# Autodesk Inventor assembly: Sestava
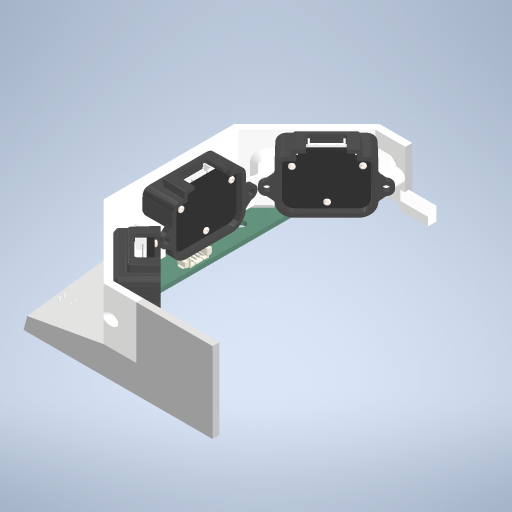
[picture p0: Inventor's stored thumbnail of the model, 512x512]
Saved by Autodesk Inventor 2024 (Build 280153000, 153)
## iProperties
Created: 2024-01-31
Part Number: Sestava
Document SubType Name: Assembly
Designer: Simak
Author: Simak
## Documents named in this file (5)
- C:\Users\Simak\OneDrive\Dokumenty\GitHub\RoboCop\- 3D -\_wip\Sestava.iam
- C:\Users\Simak\OneDrive\Dokumenty\GitHub\RoboCop\- 3D -\_wip\new_plech.ipt
- C:\Users\Simak\OneDrive\Dokumenty\GitHub\RoboCop\- 3D -\archive\TF-Luna_holder_v1\Sestava TF-Luna a držáku.iam
- C:\Users\Simak\OneDrive\Dokumenty\GitHub\RoboCop\- 3D -\PCBs\QRE MiniBoards\QRE MiniBoards\QRE_MiniBoards_Board.iam
- C:\Users\Simak\OneDrive\Dokumenty\GitHub\RoboCop\- 3D -\_wip\body.ipt
## Components (4 placed, 4 different names)
1. new_plech:1 — Proti sobě:2, Stejný směr:1, Proti sobě:3, Stejný směr:2, Vložit:1, Proti sobě:4, Stejný směr:3, Stejný směr:4
2. Sestava TF-Luna a držáku:1 [sub-assembly] — Proti sobě:2, Stejný směr:1, Proti sobě:5, Proti sobě:6
3. QRE_MiniBoards_Board:1 [sub-assembly] — Proti sobě:3, Stejný směr:2, Vložit:1
4. body:1 — Proti sobě:4, Stejný směr:3, Stejný směr:4, Proti sobě:5, Proti sobě:6
## Relationships (10: Mate 5, Flush 4, Insert 1)
- Proti sobě:2 [Mate]: new_plech:1 ↔ Sestava TF-Luna a držáku:1
- Stejný směr:1 [Flush]: new_plech:1 ↔ Sestava TF-Luna a držáku:1
- Proti sobě:3 [Mate] (1 mm): new_plech:1 ↔ QRE_MiniBoards_Board:1
- Stejný směr:2 [Flush] (4.75 mm): new_plech:1 ↔ QRE_MiniBoards_Board:1
- Vložit:1 [Insert]: new_plech:1 ↔ QRE_MiniBoards_Board:1
- Proti sobě:4 [Mate]: new_plech:1 ↔ body:1
- Stejný směr:3 [Flush]: new_plech:1 ↔ body:1
- Stejný směr:4 [Flush]: new_plech:1 ↔ body:1
- Proti sobě:5 [Mate]: Sestava TF-Luna a držáku:1 ↔ body:1
- Proti sobě:6 [Mate]: Sestava TF-Luna a držáku:1 ↔ body:1
